# Autodesk Inventor assembly: Electrode_assembly_v6
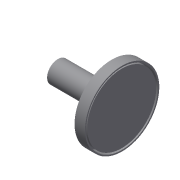
[picture p0: Inventor's stored thumbnail of the model, 180x180]
Saved by Autodesk Inventor 2015 (Build 190159000, 159)
## iProperties
Created: 2012-06-12
Part Number: Electrode_assembly_v6
Document SubType Name: Assembly
Designer: Breckenridge2 User
Author: Breckenridge2 User
## Documents named in this file (4)
- D:\kananovich\personal\d\docs\forWork\plasma\equipment\drafts\chambers\topf\kudaTopf\kuda3D\Electrode_assembly_v6.iam
- D:\kananovich\personal\d\docs\forWork\plasma\equipment\drafts\chambers\topf\kudaTopf\Electrode_v_1.ipt
- D:\kananovich\personal\d\docs\forWork\plasma\equipment\drafts\chambers\topf\kudaTopf\Teflon_spacer_v_1.ipt
- D:\kananovich\personal\d\docs\forWork\plasma\equipment\drafts\chambers\topf\kudaTopf\kuda3D\Assembly1.iam
## Components (3 placed, 3 different names)
1. Electrode_v_1:1 — Insert:2
2. Teflon_spacer_v_1:1 — Insert:1, Insert:2
3. Assembly1:1 [sub-assembly] — Insert:1
## Relationships (2: Insert 2)
- Insert:1: Teflon_spacer_v_1:1 ↔ Assembly1:1
- Insert:2: Electrode_v_1:1 ↔ Teflon_spacer_v_1:1
